# Autodesk Inventor assembly: levels
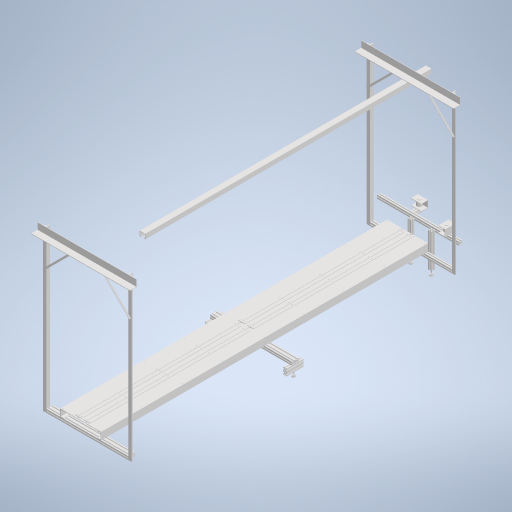
[picture p0: Inventor's stored thumbnail of the model, 512x512]
Saved by Autodesk Inventor 2023 (Build 270158030, 158C)
## iProperties
Created: 2023-02-18
Part Number: levels
Document SubType Name: Assembly
Designer: jeremyy
Author: jeremyy
## Documents named in this file (3)
- \\andrew.ad.cmu.edu\users\users1\jeremyy\Documents\Inventor\CMU Bridge\New folder\levels.iam
- \\andrew.ad.cmu.edu\users\users1\jeremyy\Documents\Inventor\CMU Bridge\New folder\Section 1.iam
- \\andrew.ad.cmu.edu\users\users1\jeremyy\Documents\Inventor\CMU Bridge\New folder\LongStrut84Sec1.ipt
## Components (2 placed, 2 different names)
1. Section 1:1 [sub-assembly] — Mate:1, Mate:2, Flush:1
2. LongStrut84Sec1:1 — Mate:1, Mate:2, Flush:1
## Relationships (3: Mate 2, Flush 1)
- Mate:1: Section 1:1 ↔ LongStrut84Sec1:1
- Mate:2 (279.4 mm): Section 1:1 ↔ LongStrut84Sec1:1
- Flush:1 (-127 mm): Section 1:1 ↔ LongStrut84Sec1:1
